# Autodesk Inventor assembly: Baugruppe1
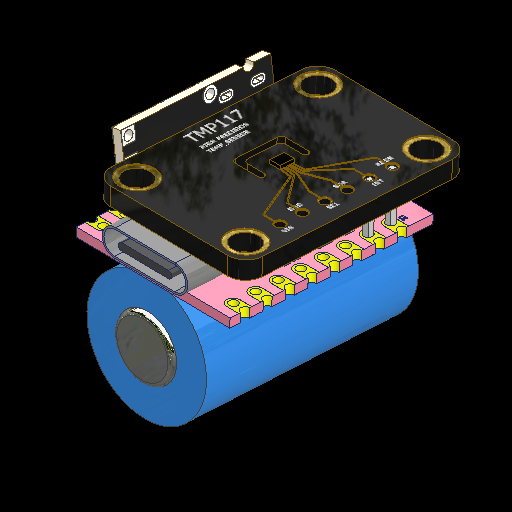
[picture p0: Inventor's stored thumbnail of the model, 512x512]
Saved by Autodesk Inventor 2027.1 (Build 311270010, 270A)
## iProperties
Created: 2026-10-09
Part Number: Baugruppe1
Document SubType Name: Assembly
Designer: josia
Author: josia
## Documents named in this file (6)
- C:\Users\josia\OneDrive\Desktop\Projekte\TemperaturSensor\tmp117_Temp_Sensor\Temp_Sensor.iam
- C:\Users\josia\OneDrive\Desktop\Projekte\TemperaturSensor\tmp117_Temp_Sensor\Verschiedene_ESP32_C3_Super_Mini_3DModele\ESP32 C3 Super mini (PINK)\ESP32 C3 Super mini (PINK).ipt
- C:\Users\josia\OneDrive\Desktop\Projekte\TemperaturSensor\tmp117_Temp_Sensor\Temp_Basis_Platte.ipt
- C:\Users\josia\OneDrive\Desktop\Projekte\TemperaturSensor\tmp117_Temp_Sensor\Pin_7mm.ipt
- C:\Users\josia\OneDrive\Desktop\Projekte\TemperaturSensor\tmp117_Temp_Sensor\charging-module-tp4057-mini-1\Charging Module TP4057 Mini\Charging Module TP4057 Mini.iam
- C:\Users\josia\OneDrive\Desktop\Projekte\TemperaturSensor\tmp117_Temp_Sensor\Li-Ion 14250.ipt
## Components (6 placed, 5 different names)
1. ESP32 C3 Super mini (PINK):1 — Passend:1, Passend:2, Winkel:1, Fluchtend:3, Fluchtend:4, Tangential:1, Fluchtend:5, Passend:6
2. Temp_Basis_Platte:1 — Passend:1, Passend:3, Passend:4, Fluchtend:1, Fluchtend:2, Passend:5, Fluchtend:4
3. Pin_7mm:1 — Passend:4, Fluchtend:1
4. Pin_7mm:2 — Passend:2, Passend:3, Fluchtend:2
5. Charging Module TP4057 Mini:1 [sub-assembly] — Winkel:1, Fluchtend:3, Passend:5
6. Li-Ion 14250:1 — Tangential:1, Fluchtend:5, Passend:6
## Relationships (13: Mate 6, Flush 5, Angle 1, Tangent 1)
- Passend:1 [Mate] (3.5 mm): ESP32 C3 Super mini (PINK):1 ↔ Temp_Basis_Platte:1
- Passend:2 [Mate]: ESP32 C3 Super mini (PINK):1 ↔ Pin_7mm:2
- Passend:3 [Mate]: Temp_Basis_Platte:1 ↔ Pin_7mm:2
- Passend:4 [Mate]: Temp_Basis_Platte:1 ↔ Pin_7mm:1
- Fluchtend:1 [Flush]: Temp_Basis_Platte:1 ↔ Pin_7mm:1
- Fluchtend:2 [Flush]: Temp_Basis_Platte:1 ↔ Pin_7mm:2
- Winkel:1 [Angle] (-10 deg): ESP32 C3 Super mini (PINK):1 ↔ Charging Module TP4057 Mini:1
- Fluchtend:3 [Flush]: ESP32 C3 Super mini (PINK):1 ↔ Charging Module TP4057 Mini:1
- Passend:5 [Mate]: Temp_Basis_Platte:1 ↔ Charging Module TP4057 Mini:1
- Fluchtend:4 [Flush]: ESP32 C3 Super mini (PINK):1 ↔ Temp_Basis_Platte:1
- Tangential:1: ESP32 C3 Super mini (PINK):1 ↔ Li-Ion 14250:1
- Fluchtend:5 [Flush] (-2 mm): ESP32 C3 Super mini (PINK):1 ↔ Li-Ion 14250:1
- Passend:6 [Mate] (-10 mm): ESP32 C3 Super mini (PINK):1 ↔ Li-Ion 14250:1
